# Autodesk Inventor assembly: Elevator
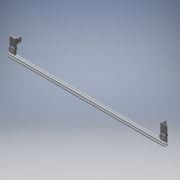
[picture p0: Inventor's stored thumbnail of the model, 180x180]
Saved by Autodesk Inventor 2017 (Build 210142000, 142)
## iProperties
Created: 2016-12-12
Part Number: Elevator
Document SubType Name: Assembly
Designer: umr
Mass: 2299.93 g
Surface Area: 5139.57 cm^2
Volume: 605.03 cm^3
Density: 3.80135 g/cm^3
Author: umr
## Documents named in this file (10)
- D:\SeniorProject\Models2\Gantry\GantryUp.iam
- D:\SeniorProject\Models2\Gantry\M5 Screw with Tee Nut.iam
- D:\SeniorProject\Models2\Gantry\DriverElevatorConnection.ipt
- D:\SeniorProject\Models2\Gantry\L_Fixer2.ipt
- D:\SeniorProject\Models2\Gantry\Tee Nut With headless screw.iam
- D:\SeniorProject\Models2\Gantry\HeaderTrack.ipt
- D:\SeniorProject\Models2\Gantry\M5 Screw with Tee Nut_MIR.iam
- D:\SeniorProject\Models2\Gantry\DriverElevatorConnection_MIR.ipt
- D:\SeniorProject\Models2\Gantry\L_Fixer2_MIR.ipt
- D:\SeniorProject\Models2\Gantry\PowerScrewNut.ipt
## Components (15 placed, 9 different names)
1. DriverElevatorConnection:1 — Mate:50, Mate:51, Mate:52, Mate:75, Mate:76, Mate:77, Mate:78, Flush:1, Mate:176, Mate:177
2. L_Fixer2:1 — Mate:50, Mate:51, Mate:52, Mate:59, Mate:60, Mate:61, Mate:62
3. M5 Screw with Tee Nut:13 [sub-assembly] — Mate:59, Mate:62
4. M5 Screw with Tee Nut:14 [sub-assembly] — Mate:60, Mate:61
5. Tee Nut With headless screw:1 [sub-assembly] — Mate:76, Mate:78, Mate:81
6. Tee Nut With headless screw:2 [sub-assembly] — Mate:75, Mate:77, Mate:79, Mate:80
7. HeaderTrack:1 — Mate:79, Mate:80, Mate:81, Flush:1, Mate:169, Mate:170, Mate:171, Mate:172
8. DriverElevatorConnection_MIR:1 — Mate:144, Mate:145, Mate:146, Mate:173, Mate:174, Mate:175, Mate:178
9. L_Fixer2_MIR:1 — Mate:144, Mate:145, Mate:146, Mate:161, Mate:162, Mate:164, Mate:165
10. M5 Screw with Tee Nut_MIR:13 [sub-assembly] — Mate:161, Mate:162
11. M5 Screw with Tee Nut_MIR:14 [sub-assembly] — Mate:164, Mate:165
12. Tee Nut With headless screw:3 [sub-assembly] — Mate:169, Mate:172, Mate:174
13. Tee Nut With headless screw:4 [sub-assembly] — Mate:170, Mate:171, Mate:173
14. PowerScrewNut:1 — Mate:175, Mate:178
15. PowerScrewNut:2 — Mate:176, Mate:177
## Relationships (32: Mate 31, Flush 1)
- Mate:50: DriverElevatorConnection:1 ↔ L_Fixer2:1
- Mate:51: DriverElevatorConnection:1 ↔ L_Fixer2:1
- Mate:52: DriverElevatorConnection:1 ↔ L_Fixer2:1
- Mate:59: L_Fixer2:1 ↔ M5 Screw with Tee Nut:13
- Mate:60: L_Fixer2:1 ↔ M5 Screw with Tee Nut:14
- Mate:61: L_Fixer2:1 ↔ M5 Screw with Tee Nut:14
- Mate:62: L_Fixer2:1 ↔ M5 Screw with Tee Nut:13
- Mate:75: DriverElevatorConnection:1 ↔ Tee Nut With headless screw:2
- Mate:76: DriverElevatorConnection:1 ↔ Tee Nut With headless screw:1
- Mate:77: DriverElevatorConnection:1 ↔ Tee Nut With headless screw:2
- Mate:78: DriverElevatorConnection:1 ↔ Tee Nut With headless screw:1
- Mate:79: Tee Nut With headless screw:2 ↔ HeaderTrack:1
- Mate:80: Tee Nut With headless screw:2 ↔ HeaderTrack:1
- Mate:81: Tee Nut With headless screw:1 ↔ HeaderTrack:1
- Flush:1: DriverElevatorConnection:1 ↔ HeaderTrack:1
- Mate:144: DriverElevatorConnection_MIR:1 ↔ L_Fixer2_MIR:1
- Mate:145: DriverElevatorConnection_MIR:1 ↔ L_Fixer2_MIR:1
- Mate:146: DriverElevatorConnection_MIR:1 ↔ L_Fixer2_MIR:1
- Mate:161: L_Fixer2_MIR:1 ↔ M5 Screw with Tee Nut_MIR:13
- Mate:162: L_Fixer2_MIR:1 ↔ M5 Screw with Tee Nut_MIR:13
- Mate:164: L_Fixer2_MIR:1 ↔ M5 Screw with Tee Nut_MIR:14
- Mate:165: L_Fixer2_MIR:1 ↔ M5 Screw with Tee Nut_MIR:14
- Mate:169 (1 mm): HeaderTrack:1 ↔ Tee Nut With headless screw:3
- Mate:170: HeaderTrack:1 ↔ Tee Nut With headless screw:4
- Mate:171 (0.5 mm): HeaderTrack:1 ↔ Tee Nut With headless screw:4
- Mate:172 (0.5 mm): HeaderTrack:1 ↔ Tee Nut With headless screw:3
- Mate:173: DriverElevatorConnection_MIR:1 ↔ Tee Nut With headless screw:4
- Mate:174: DriverElevatorConnection_MIR:1 ↔ Tee Nut With headless screw:3
- Mate:175: DriverElevatorConnection_MIR:1 ↔ PowerScrewNut:1
- Mate:176: DriverElevatorConnection:1 ↔ PowerScrewNut:2
- Mate:177: DriverElevatorConnection:1 ↔ PowerScrewNut:2
- Mate:178: DriverElevatorConnection_MIR:1 ↔ PowerScrewNut:1
